# Autodesk Inventor assembly: gear40
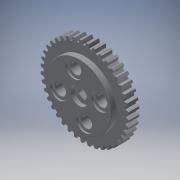
[picture p0: Inventor's stored thumbnail of the model, 180x180]
Saved by Autodesk Inventor 2019 (Build 230136000, 136)
## iProperties
Created: 2019-01-24
Part Number: gear40
Document SubType Name: Assembly
Designer: Varga Daniel
Author: Varga Daniel
## Documents named in this file (3)
- C:\!_Dani\!_cloud\OneDrive\!_munka\Revolution\RevvyDemoKit\Structural parts\Demo parts\Gears\gear40.iam
- C:\!_Dani\!_cloud\OneDrive\!_munka\Revolution\RevvyDemoKit\Structural parts\Demo parts\Gears\gear40.ipt
- C:\!_Dani\!_cloud\OneDrive\!_munka\Revolution\RevvyDemoKit\Structural parts\Demo parts\Gears\gear_collar.ipt
## Components (3 placed, 2 different names)
1. gear_collar:1 — Flush:1, Flush:2, Angle:1
2. gear40:1 — Mate:3, Angle:1
3. gear_collar:2 — Flush:1, Flush:2, Mate:3
## Relationships (4: Flush 2, Mate 1, Angle 1)
- Flush:1: gear_collar:1 ↔ gear_collar:2
- Flush:2: gear_collar:1 ↔ gear_collar:2
- Mate:3: gear40:1 ↔ gear_collar:2
- Angle:1 (0 deg): gear_collar:1 ↔ gear40:1
